# Autodesk Inventor assembly: Assembly1
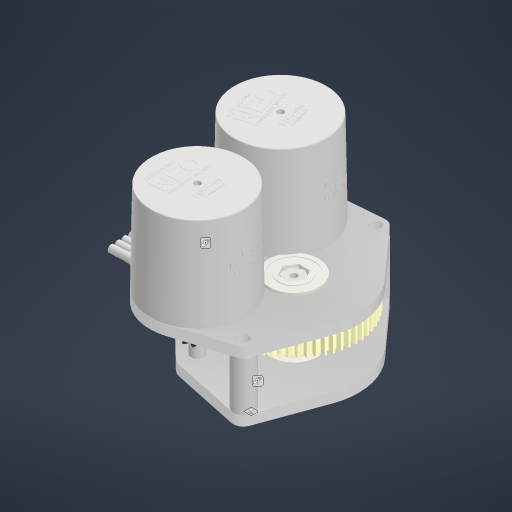
[picture p0: Inventor's stored thumbnail of the model, 512x512]
Saved by Autodesk Inventor 2024.3 (Build 283343000, 343)
## iProperties
Created: 2024-11-01
Part Number: Assembly1
Document SubType Name: Assembly
Designer: kaito
Author: kaito
## Documents named in this file (9)
- C:\Users\kaito\OneDrive\Documents\GitHub\1622-2024-Assignments\Kaito Kubota-Valme\Gearbox 2 v.2\Assembly1.iam
- C:\Users\kaito\OneDrive\Documents\GitHub\1622-2024-Assignments\Kaito Kubota-Valme\Gearbox 2 v.2\Bottom Plate.ipt
- C:\Users\kaito\OneDrive\Documents\GitHub\1622-2024-Assignments\Kaito Kubota-Valme\Gearbox 2 v.2\Part1.ipt
- C:\Users\kaito\OneDrive\Desktop\COTS Library\Motion\Bearings\COTS_WCP-0783_1.125ODHexBearing.ipt
- C:\Users\kaito\OneDrive\Desktop\COTS Library\Motion\Gears\Motor Gears\COTS_217-6334_10T20DPMotorGear.ipt
- C:\Users\kaito\Downloads\REV-21-1650-V1.1\REV-21-1650-V1.1\REV-21-1650-V1.1.ipt
- C:\Users\kaito\OneDrive\Documents\GitHub\1622-2024-Assignments\Kaito Kubota-Valme\Gearbox 2 v.2\Standoff.ipt
- C:\Users\kaito\OneDrive\Documents\GitHub\1622-2024-Assignments\Kaito Kubota-Valme\Gearbox 2 v.2\Hex Shaft.ipt
- C:\Users\kaito\Downloads\WCP-0720 (2)\WCP-0720 (2)\WCP-0720 (2).ipt
## Components (13 placed, 8 different names)
1. Bottom Plate:1 — Mate:5, Mate:15, Mate:16, Mate:17, Mate:19, Mate:21, Mate:24, Mate:25
2. Part1:1 — Mate:2, Mate:3, Mate:5, Mate:6, Mate:7, Mate:8, Mate:9, Mate:10, Mate:12, Mate:14, Mate:17, Mate:18, Mate:20, Mate:22, Mate:23
3. COTS_WCP-0783_1.125ODHexBearing:1 — Mate:2, Mate:3, Mate:28
4. COTS_217-6334_10T20DPMotorGear:1 — Mate:13, Mate:14
5. COTS_217-6334_10T20DPMotorGear:2 — Mate:11, Mate:12
6. REV-21-1650-V1.1:1 — Mate:6, Mate:7, Mate:8, Mate:11
7. REV-21-1650-V1.1:2 — Mate:9, Mate:10, Mate:13, Mate:23
8. Standoff:1 — Mate:21, Mate:22
9. Standoff:2 — Mate:15, Mate:16, Mate:18
10. Standoff:3 — Mate:19, Mate:20
11. Hex Shaft:1 — Mate:26, Flush:1, Mate:27
12. COTS_WCP-0783_1.125ODHexBearing:2 — Mate:24, Mate:25, Mate:26, Flush:1
13. WCP-0720 (2):1 — Mate:27, Mate:28
## Relationships (27: Mate 26, Flush 1)
- Mate:2: Part1:1 ↔ COTS_WCP-0783_1.125ODHexBearing:1
- Mate:3: Part1:1 ↔ COTS_WCP-0783_1.125ODHexBearing:1
- Mate:5: Bottom Plate:1 ↔ Part1:1
- Mate:6: Part1:1 ↔ REV-21-1650-V1.1:1
- Mate:7: Part1:1 ↔ REV-21-1650-V1.1:1
- Mate:8: Part1:1 ↔ REV-21-1650-V1.1:1
- Mate:9: Part1:1 ↔ REV-21-1650-V1.1:2
- Mate:10: Part1:1 ↔ REV-21-1650-V1.1:2
- Mate:11: COTS_217-6334_10T20DPMotorGear:2 ↔ REV-21-1650-V1.1:1
- Mate:12: Part1:1 ↔ COTS_217-6334_10T20DPMotorGear:2
- Mate:13: COTS_217-6334_10T20DPMotorGear:1 ↔ REV-21-1650-V1.1:2
- Mate:14: Part1:1 ↔ COTS_217-6334_10T20DPMotorGear:1
- Mate:15: Bottom Plate:1 ↔ Standoff:2
- Mate:16: Bottom Plate:1 ↔ Standoff:2
- Mate:17: Bottom Plate:1 ↔ Part1:1
- Mate:18: Part1:1 ↔ Standoff:2
- Mate:19: Bottom Plate:1 ↔ Standoff:3
- Mate:20: Part1:1 ↔ Standoff:3
- Mate:21: Bottom Plate:1 ↔ Standoff:1
- Mate:22: Part1:1 ↔ Standoff:1
- Mate:23: Part1:1 ↔ REV-21-1650-V1.1:2
- Mate:24: Bottom Plate:1 ↔ COTS_WCP-0783_1.125ODHexBearing:2
- Mate:25: Bottom Plate:1 ↔ COTS_WCP-0783_1.125ODHexBearing:2
- Mate:26: Hex Shaft:1 ↔ COTS_WCP-0783_1.125ODHexBearing:2
- Flush:1: Hex Shaft:1 ↔ COTS_WCP-0783_1.125ODHexBearing:2
- Mate:27: Hex Shaft:1 ↔ WCP-0720 (2):1
- Mate:28: COTS_WCP-0783_1.125ODHexBearing:1 ↔ WCP-0720 (2):1
